# Autodesk Inventor assembly: Chassis-ver9-1111-2019
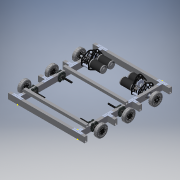
[picture p0: Inventor's stored thumbnail of the model, 180x180]
Saved by Autodesk Inventor 2018 (Build 220112000, 112)
## iProperties
Created: 2019-10-10
Part Number: Chassis-ver9-1111-2019
Document SubType Name: Assembly
Designer: JMHal
Author: JMHal
## Documents named in this file (11)
- F:\GrabCad\2019 - 2020 Off Season\TestChassis\Assembly\Chassis-ver9-1111-2019.iam
- F:\GrabCad\2019 - 2020 Off Season\TestChassis\Parts\2x1 20in Alluminum with Cal Drop.ver1-1111-2019.ipt
- F:\GrabCad\2019 - 2020 Off Season\TestChassis\Parts\2x1 20in Alluminum.ver1-1111-2019.ipt
- F:\GrabCad\2019 - 2020 Off Season\TestChassis\Parts\2x1 2in Alluminum Block.ver1-1111-2019.ipt
- F:\GrabCad\Resources\VEXpro Resources\Bearings\0.5inHexFlangedBearing(1.125inx0.313in)-1111-2016.ipt
- F:\GrabCad\Resources\VEXpro Resources\Versa Motion\VersaBlockKit-1111-2016.ipt
- F:\GrabCad\Resources\VEXpro Resources\Wheels\4 inch\4x1inTractionWheel(Tire)-1111-2016.iam
- F:\GrabCad\Resources\VEXpro Resources\Shafts\0.5inThunderHexShaft(8)-1111-2016.ipt
- F:\GrabCad\Resources\VEXpro Resources\Gearboxes\WCP SS Gearbox\SS-Gearbox.iam
- F:\GrabCad\Resources\VEXpro Resources\Gussets\ChassisGusset-1111-2016.ipt
- F:\GrabCad\2019 - 2020 Off Season\TestChassis\Parts\ElectricalBoardSupport.ver1-1111-2019.ipt
## Components (46 placed, 10 different names)
1. 2x1 20in Alluminum with Cal Drop.ver1-1111-2019:1 — Mate:31, Mate:32, Insert:7, Mate:51, Insert:8, Angle:2, Mate:53, Angle:9, Insert:17, Angle:10, Insert:19, Angle:11, Mate:60, Cylindrical:1, Angle:16, Mate:64, Flush:1, Mate:65, Mate:66, Flush:2, Flush:3, Mate:67, Flush:4, Flush:5, Mate:77, Mate:78, Flush:16, Flush:17, Mate:80, Flush:20, Flush:23, Mate:83
2. 2x1 20in Alluminum.ver1-1111-2019:1 — Mate:65, Mate:66, Flush:2, Flush:3, Mate:68, Mate:72, Mate:81, Flush:22, Mate:82, Flush:24, Mate:84
3. 2x1 20in Alluminum with Cal Drop.ver1-1111-2019:2 — Insert:4, Insert:5, Angle:7, Angle:8, Insert:23, Angle:13, Insert:25, Angle:14, Rotational:1, Angle:17, Flush:6, Flush:7, Mate:70, Flush:8, Mate:73, Mate:74, Flush:9, Flush:10, Flush:13, Flush:18, Flush:25, Flush:26, Mate:85, Flush:27
4. 2x1 20in Alluminum.ver1-1111-2019:2 — Mate:67, Flush:4, Flush:5, Mate:69, Flush:6, Flush:7, Mate:71, Mate:73, Mate:79, Flush:19, Flush:21
5. 0.5inThunderHexShaft(8)-1111-2016:1 — Cylindrical:2, Rotational:9
6. SS-Gearbox:1 [sub-assembly] — Rotational:1, Angle:17, Rotational:2
7. SS-Gearbox:2 [sub-assembly] — Mate:60, Cylindrical:1, Angle:16, Cylindrical:11, Mate:61
8. 0.5inThunderHexShaft(8)-1111-2016:2 — Cylindrical:3, Rotational:8
9. 0.5inThunderHexShaft(8)-1111-2016:3 — Rotational:16, Rotational:4
10. 0.5inThunderHexShaft(8)-1111-2016:4 — Rotational:14, Rotational:13
11. ChassisGusset-1111-2016:1 — Mate:76, Flush:12, Flush:13
12. ChassisGusset-1111-2016:2 — Mate:75, Flush:10, Flush:11
13. ChassisGusset-1111-2016:3 — Mate:78, Flush:14, Flush:17
14. ChassisGusset-1111-2016:4 — Mate:77, Flush:15, Flush:16
15. ChassisGusset-1111-2016:5 — Mate:82, Flush:24, Flush:25
16. ChassisGusset-1111-2016:6 — Mate:81, Flush:22, Flush:23
17. ChassisGusset-1111-2016:7 — Mate:80, Flush:20, Flush:21
18. ChassisGusset-1111-2016:8 — Mate:79, Flush:18, Flush:19
19. ElectricalBoardSupport.ver1-1111-2019:1 — Mate:83, Flush:26, Mate:84, Mate:86
20. ElectricalBoardSupport.ver1-1111-2019:2 — Mate:85, Flush:27, Mate:86
21. 0.5inHexFlangedBearing(1.125inx0.313in)-1111-2016:20 — Rotational:14
22. 0.5inHexFlangedBearing(1.125inx0.313in)-1111-2016:19 — Rotational:16
23. 0.5inHexFlangedBearing(1.125inx0.313in)-1111-2016:6 — Insert:4, Mate:46, Mate:47
24. 0.5inHexFlangedBearing(1.125inx0.313in)-1111-2016:7 — Insert:5, Mate:48, Mate:49
25. 0.5inHexFlangedBearing(1.125inx0.313in)-1111-2016:17 — Insert:19, Cylindrical:3
26. 0.5inHexFlangedBearing(1.125inx0.313in)-1111-2016:16 — Insert:16, Insert:17, Cylindrical:2
27. 0.5inHexFlangedBearing(1.125inx0.313in)-1111-2016:9 — Insert:7, Mate:50, Mate:63
28. 0.5inHexFlangedBearing(1.125inx0.313in)-1111-2016:10 — Insert:8, Mate:52, Mate:62
29. 2x1 2in Alluminum Block.ver1-1111-2019:5 — Mate:31, Mate:32, Mate:69, Flush:15
30. 2x1 2in Alluminum Block.ver1-1111-2019:6 — Mate:64, Flush:1, Mate:68, Flush:14
31. 2x1 2in Alluminum Block.ver1-1111-2019:7 — Mate:72, Mate:74, Flush:9, Mate:75, Flush:11
32. 2x1 2in Alluminum Block.ver1-1111-2019:8 — Mate:70, Flush:8, Mate:71, Mate:76, Flush:12
33. VersaBlockKit-1111-2016:2 — Mate:46, Mate:47, Angle:8
34. VersaBlockKit-1111-2016:3 — Mate:48, Mate:49, Angle:7
35. VersaBlockKit-1111-2016:5 — Mate:50, Mate:51, Angle:2
36. VersaBlockKit-1111-2016:6 — Mate:52, Mate:53, Angle:9
37. VersaBlockKit-1111-2016:8 — Insert:16, Angle:10
38. VersaBlockKit-1111-2016:9 — Angle:11
39. VersaBlockKit-1111-2016:11 — Insert:23, Angle:13
40. VersaBlockKit-1111-2016:12 — Insert:25, Angle:14
41. 4x1inTractionWheel(Tire)-1111-2016:1 [sub-assembly] — Rotational:2
42. 4x1inTractionWheel(Tire)-1111-2016:2 [sub-assembly] — Rotational:13
43. 4x1inTractionWheel(Tire)-1111-2016:3 [sub-assembly] — Rotational:4
44. 4x1inTractionWheel(Tire)-1111-2016:4 [sub-assembly] — Cylindrical:11, Mate:61
45. 4x1inTractionWheel(Tire)-1111-2016:5 [sub-assembly] — Rotational:9, Mate:63
46. 4x1inTractionWheel(Tire)-1111-2016:6 [sub-assembly] — Rotational:8, Mate:62
## Relationships (102: Mate 41, Flush 27, Insert 12, Angle 10, RevoluteJoint 8, CylindricalJoint 4)
- Mate:31: 2x1 20in Alluminum with Cal Drop.ver1-1111-2019:1 ↔ 2x1 2in Alluminum Block.ver1-1111-2019:5
- Mate:32: 2x1 20in Alluminum with Cal Drop.ver1-1111-2019:1 ↔ 2x1 2in Alluminum Block.ver1-1111-2019:5
- Insert:4: 2x1 20in Alluminum with Cal Drop.ver1-1111-2019:2 ↔ 0.5inHexFlangedBearing(1.125inx0.313in)-1111-2016:6
- Mate:46: 0.5inHexFlangedBearing(1.125inx0.313in)-1111-2016:6 ↔ VersaBlockKit-1111-2016:2
- Mate:47: 0.5inHexFlangedBearing(1.125inx0.313in)-1111-2016:6 ↔ VersaBlockKit-1111-2016:2
- Insert:5: 2x1 20in Alluminum with Cal Drop.ver1-1111-2019:2 ↔ 0.5inHexFlangedBearing(1.125inx0.313in)-1111-2016:7
- Mate:48: 0.5inHexFlangedBearing(1.125inx0.313in)-1111-2016:7 ↔ VersaBlockKit-1111-2016:3
- Mate:49: 0.5inHexFlangedBearing(1.125inx0.313in)-1111-2016:7 ↔ VersaBlockKit-1111-2016:3
- Insert:7: 2x1 20in Alluminum with Cal Drop.ver1-1111-2019:1 ↔ 0.5inHexFlangedBearing(1.125inx0.313in)-1111-2016:9
- Mate:50: 0.5inHexFlangedBearing(1.125inx0.313in)-1111-2016:9 ↔ VersaBlockKit-1111-2016:5
- Mate:51: 2x1 20in Alluminum with Cal Drop.ver1-1111-2019:1 ↔ VersaBlockKit-1111-2016:5
- Insert:8: 2x1 20in Alluminum with Cal Drop.ver1-1111-2019:1 ↔ 0.5inHexFlangedBearing(1.125inx0.313in)-1111-2016:10
- Angle:2 (0 deg): 2x1 20in Alluminum with Cal Drop.ver1-1111-2019:1 ↔ VersaBlockKit-1111-2016:5
- Angle:7 (0 deg): 2x1 20in Alluminum with Cal Drop.ver1-1111-2019:2 ↔ VersaBlockKit-1111-2016:3
- Angle:8 (0 deg): 2x1 20in Alluminum with Cal Drop.ver1-1111-2019:2 ↔ VersaBlockKit-1111-2016:2
- Mate:52: 0.5inHexFlangedBearing(1.125inx0.313in)-1111-2016:10 ↔ VersaBlockKit-1111-2016:6
- Mate:53: 2x1 20in Alluminum with Cal Drop.ver1-1111-2019:1 ↔ VersaBlockKit-1111-2016:6
- Angle:9 (0 deg): 2x1 20in Alluminum with Cal Drop.ver1-1111-2019:1 ↔ VersaBlockKit-1111-2016:6
- [Mate]: 0.5inHexFlangedBearing(1.125inx0.313in)-1111-2016:16 ↔ VersaBlockKit-1111-2016:8
- Insert:16: 0.5inHexFlangedBearing(1.125inx0.313in)-1111-2016:16 ↔ VersaBlockKit-1111-2016:8
- Insert:17: 2x1 20in Alluminum with Cal Drop.ver1-1111-2019:1 ↔ 0.5inHexFlangedBearing(1.125inx0.313in)-1111-2016:16
- Angle:10 (0 deg): 2x1 20in Alluminum with Cal Drop.ver1-1111-2019:1 ↔ VersaBlockKit-1111-2016:8
- [Mate]: 0.5inHexFlangedBearing(1.125inx0.313in)-1111-2016:17 ↔ VersaBlockKit-1111-2016:9
- [Insert]: 0.5inHexFlangedBearing(1.125inx0.313in)-1111-2016:17 ↔ VersaBlockKit-1111-2016:9
- Insert:19: 2x1 20in Alluminum with Cal Drop.ver1-1111-2019:1 ↔ 0.5inHexFlangedBearing(1.125inx0.313in)-1111-2016:17
- Angle:11 (0 deg): 2x1 20in Alluminum with Cal Drop.ver1-1111-2019:1 ↔ VersaBlockKit-1111-2016:9
- [Mate]: 0.5inHexFlangedBearing(1.125inx0.313in)-1111-2016:19 ↔ VersaBlockKit-1111-2016:11
- [Insert]: 0.5inHexFlangedBearing(1.125inx0.313in)-1111-2016:19 ↔ VersaBlockKit-1111-2016:11
- Insert:23: 2x1 20in Alluminum with Cal Drop.ver1-1111-2019:2 ↔ VersaBlockKit-1111-2016:11
- Angle:13 (0 deg): 2x1 20in Alluminum with Cal Drop.ver1-1111-2019:2 ↔ VersaBlockKit-1111-2016:11
- [Mate]: 0.5inHexFlangedBearing(1.125inx0.313in)-1111-2016:20 ↔ VersaBlockKit-1111-2016:12
- [Insert]: 0.5inHexFlangedBearing(1.125inx0.313in)-1111-2016:20 ↔ VersaBlockKit-1111-2016:12
- Insert:25: 2x1 20in Alluminum with Cal Drop.ver1-1111-2019:2 ↔ VersaBlockKit-1111-2016:12
- Angle:14 (0 deg): 2x1 20in Alluminum with Cal Drop.ver1-1111-2019:2 ↔ VersaBlockKit-1111-2016:12
- Mate:60: 2x1 20in Alluminum with Cal Drop.ver1-1111-2019:1 ↔ SS-Gearbox:2
- Cylindrical:1: 2x1 20in Alluminum with Cal Drop.ver1-1111-2019:1 ↔ SS-Gearbox:2
- Cylindrical:2: 0.5inThunderHexShaft(8)-1111-2016:1 ↔ 0.5inHexFlangedBearing(1.125inx0.313in)-1111-2016:16
- Cylindrical:3: 0.5inThunderHexShaft(8)-1111-2016:2 ↔ 0.5inHexFlangedBearing(1.125inx0.313in)-1111-2016:17
- Rotational:16 [RevoluteJoint] (91.44 mm): 0.5inThunderHexShaft(8)-1111-2016:3 ↔ 0.5inHexFlangedBearing(1.125inx0.313in)-1111-2016:19
- Rotational:14 [RevoluteJoint] (91.44 mm): 0.5inThunderHexShaft(8)-1111-2016:4 ↔ 0.5inHexFlangedBearing(1.125inx0.313in)-1111-2016:20
- Angle:16 (90 deg): 2x1 20in Alluminum with Cal Drop.ver1-1111-2019:1 ↔ SS-Gearbox:2
- Rotational:1 [RevoluteJoint]: 2x1 20in Alluminum with Cal Drop.ver1-1111-2019:2 ↔ SS-Gearbox:1
- Angle:17 (90 deg): 2x1 20in Alluminum with Cal Drop.ver1-1111-2019:2 ↔ SS-Gearbox:1
- Rotational:2 [RevoluteJoint]: SS-Gearbox:1 ↔ 4x1inTractionWheel(Tire)-1111-2016:1
- Rotational:4 [RevoluteJoint]: 0.5inThunderHexShaft(8)-1111-2016:3 ↔ 4x1inTractionWheel(Tire)-1111-2016:3
- Cylindrical:11: SS-Gearbox:2 ↔ 4x1inTractionWheel(Tire)-1111-2016:4
- Rotational:9 [RevoluteJoint]: 0.5inThunderHexShaft(8)-1111-2016:1 ↔ 4x1inTractionWheel(Tire)-1111-2016:5
- Mate:61 (-74.93 mm): SS-Gearbox:2 ↔ 4x1inTractionWheel(Tire)-1111-2016:4
- Rotational:8 [RevoluteJoint]: 0.5inThunderHexShaft(8)-1111-2016:2 ↔ 4x1inTractionWheel(Tire)-1111-2016:6
- Mate:62 (-71.12 mm): 0.5inHexFlangedBearing(1.125inx0.313in)-1111-2016:10 ↔ 4x1inTractionWheel(Tire)-1111-2016:6
- Mate:63 (-74.422 mm): 0.5inHexFlangedBearing(1.125inx0.313in)-1111-2016:9 ↔ 4x1inTractionWheel(Tire)-1111-2016:5
- Rotational:13 [RevoluteJoint]: 0.5inThunderHexShaft(8)-1111-2016:4 ↔ 4x1inTractionWheel(Tire)-1111-2016:2
- Mate:64: 2x1 20in Alluminum with Cal Drop.ver1-1111-2019:1 ↔ 2x1 2in Alluminum Block.ver1-1111-2019:6
- Flush:1: 2x1 20in Alluminum with Cal Drop.ver1-1111-2019:1 ↔ 2x1 2in Alluminum Block.ver1-1111-2019:6
- Mate:65: 2x1 20in Alluminum with Cal Drop.ver1-1111-2019:1 ↔ 2x1 20in Alluminum.ver1-1111-2019:1
- Mate:66: 2x1 20in Alluminum with Cal Drop.ver1-1111-2019:1 ↔ 2x1 20in Alluminum.ver1-1111-2019:1
- Flush:2: 2x1 20in Alluminum with Cal Drop.ver1-1111-2019:1 ↔ 2x1 20in Alluminum.ver1-1111-2019:1
- Flush:3 (63.5 mm): 2x1 20in Alluminum with Cal Drop.ver1-1111-2019:1 ↔ 2x1 20in Alluminum.ver1-1111-2019:1
- Mate:67: 2x1 20in Alluminum with Cal Drop.ver1-1111-2019:1 ↔ 2x1 20in Alluminum.ver1-1111-2019:2
- Flush:4: 2x1 20in Alluminum with Cal Drop.ver1-1111-2019:1 ↔ 2x1 20in Alluminum.ver1-1111-2019:2
- Flush:5 (-63.5 mm): 2x1 20in Alluminum with Cal Drop.ver1-1111-2019:1 ↔ 2x1 20in Alluminum.ver1-1111-2019:2
- Mate:68 (254 mm): 2x1 20in Alluminum.ver1-1111-2019:1 ↔ 2x1 2in Alluminum Block.ver1-1111-2019:6
- Mate:69 (254 mm): 2x1 20in Alluminum.ver1-1111-2019:2 ↔ 2x1 2in Alluminum Block.ver1-1111-2019:5
- Flush:6: 2x1 20in Alluminum with Cal Drop.ver1-1111-2019:2 ↔ 2x1 20in Alluminum.ver1-1111-2019:2
- Flush:7 (63.5 mm): 2x1 20in Alluminum with Cal Drop.ver1-1111-2019:2 ↔ 2x1 20in Alluminum.ver1-1111-2019:2
- Mate:70: 2x1 20in Alluminum with Cal Drop.ver1-1111-2019:2 ↔ 2x1 2in Alluminum Block.ver1-1111-2019:8
- Flush:8: 2x1 20in Alluminum with Cal Drop.ver1-1111-2019:2 ↔ 2x1 2in Alluminum Block.ver1-1111-2019:8
- Mate:71 (254 mm): 2x1 20in Alluminum.ver1-1111-2019:2 ↔ 2x1 2in Alluminum Block.ver1-1111-2019:8
- Mate:72 (254 mm): 2x1 20in Alluminum.ver1-1111-2019:1 ↔ 2x1 2in Alluminum Block.ver1-1111-2019:7
- Mate:73: 2x1 20in Alluminum with Cal Drop.ver1-1111-2019:2 ↔ 2x1 20in Alluminum.ver1-1111-2019:2
- Mate:74: 2x1 20in Alluminum with Cal Drop.ver1-1111-2019:2 ↔ 2x1 2in Alluminum Block.ver1-1111-2019:7
- Flush:9: 2x1 20in Alluminum with Cal Drop.ver1-1111-2019:2 ↔ 2x1 2in Alluminum Block.ver1-1111-2019:7
- Mate:75: ChassisGusset-1111-2016:2 ↔ 2x1 2in Alluminum Block.ver1-1111-2019:7
- Flush:10: 2x1 20in Alluminum with Cal Drop.ver1-1111-2019:2 ↔ ChassisGusset-1111-2016:2
- Flush:11: ChassisGusset-1111-2016:2 ↔ 2x1 2in Alluminum Block.ver1-1111-2019:7
- Mate:76: ChassisGusset-1111-2016:1 ↔ 2x1 2in Alluminum Block.ver1-1111-2019:8
- Flush:12: ChassisGusset-1111-2016:1 ↔ 2x1 2in Alluminum Block.ver1-1111-2019:8
- Flush:13: 2x1 20in Alluminum with Cal Drop.ver1-1111-2019:2 ↔ ChassisGusset-1111-2016:1
- Mate:77: 2x1 20in Alluminum with Cal Drop.ver1-1111-2019:1 ↔ ChassisGusset-1111-2016:4
- Mate:78: 2x1 20in Alluminum with Cal Drop.ver1-1111-2019:1 ↔ ChassisGusset-1111-2016:3
- Flush:14: ChassisGusset-1111-2016:3 ↔ 2x1 2in Alluminum Block.ver1-1111-2019:6
- Flush:15: ChassisGusset-1111-2016:4 ↔ 2x1 2in Alluminum Block.ver1-1111-2019:5
- Flush:16: 2x1 20in Alluminum with Cal Drop.ver1-1111-2019:1 ↔ ChassisGusset-1111-2016:4
- Flush:17: 2x1 20in Alluminum with Cal Drop.ver1-1111-2019:1 ↔ ChassisGusset-1111-2016:3
- Mate:79: 2x1 20in Alluminum.ver1-1111-2019:2 ↔ ChassisGusset-1111-2016:8
- Flush:18: 2x1 20in Alluminum with Cal Drop.ver1-1111-2019:2 ↔ ChassisGusset-1111-2016:8
- Flush:19: 2x1 20in Alluminum.ver1-1111-2019:2 ↔ ChassisGusset-1111-2016:8
- Mate:80: 2x1 20in Alluminum with Cal Drop.ver1-1111-2019:1 ↔ ChassisGusset-1111-2016:7
- Flush:20: 2x1 20in Alluminum with Cal Drop.ver1-1111-2019:1 ↔ ChassisGusset-1111-2016:7
- Flush:21: 2x1 20in Alluminum.ver1-1111-2019:2 ↔ ChassisGusset-1111-2016:7
- Mate:81: 2x1 20in Alluminum.ver1-1111-2019:1 ↔ ChassisGusset-1111-2016:6
- Flush:22: 2x1 20in Alluminum.ver1-1111-2019:1 ↔ ChassisGusset-1111-2016:6
- Flush:23: 2x1 20in Alluminum with Cal Drop.ver1-1111-2019:1 ↔ ChassisGusset-1111-2016:6
- Mate:82: 2x1 20in Alluminum.ver1-1111-2019:1 ↔ ChassisGusset-1111-2016:5
- Flush:24: 2x1 20in Alluminum.ver1-1111-2019:1 ↔ ChassisGusset-1111-2016:5
- Flush:25: 2x1 20in Alluminum with Cal Drop.ver1-1111-2019:2 ↔ ChassisGusset-1111-2016:5
- Mate:83: 2x1 20in Alluminum with Cal Drop.ver1-1111-2019:1 ↔ ElectricalBoardSupport.ver1-1111-2019:1
- Flush:26: 2x1 20in Alluminum with Cal Drop.ver1-1111-2019:2 ↔ ElectricalBoardSupport.ver1-1111-2019:1
- Mate:84 (50.8 mm): 2x1 20in Alluminum.ver1-1111-2019:1 ↔ ElectricalBoardSupport.ver1-1111-2019:1
- Mate:85: 2x1 20in Alluminum with Cal Drop.ver1-1111-2019:2 ↔ ElectricalBoardSupport.ver1-1111-2019:2
- Flush:27: 2x1 20in Alluminum with Cal Drop.ver1-1111-2019:2 ↔ ElectricalBoardSupport.ver1-1111-2019:2
- Mate:86 (342.9 mm): ElectricalBoardSupport.ver1-1111-2019:1 ↔ ElectricalBoardSupport.ver1-1111-2019:2
## Named parameters: d89_d76 = 0 mm, d93_d89_d76 = 0 mm, d94_d90 = 0 mm, d103_d89_d76 = 0 mm, d104_d90 = 0 mm, d107_d89_d76 = 0 mm, d108_d90 = 0 mm
